# Autodesk Inventor assembly: drive_parts_assembly_z
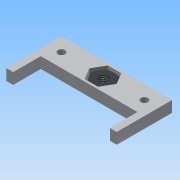
[picture p0: Inventor's stored thumbnail of the model, 180x180]
Saved by Autodesk Inventor 2015 (Build 190159000, 159)
## iProperties
Created: 2014-09-02
Part Number: drive_parts_assembly_z
Document SubType Name: Assembly
Designer: shohei
Author: shohei
## Documents named in this file (3)
- C:\Users\shohei\Documents\Inventor\PlasmaCNCrev3\Workspaces\Workspace\drive_parts_assembly_z.iam
- C:\Users\shohei\Documents\Inventor\PlasmaCNCrev3\Workspaces\Workspace\main\M8_driving_nut.ipt
- C:\Users\shohei\Documents\Inventor\PlasmaCNCrev3\Workspaces\Workspace\main\drive_support.ipt
## Components (2 placed, 2 different names)
1. M8_driving_nut:1 — Flush:1, Angle:1
2. drive_support:1 — Flush:1, Angle:1
## Relationships (2: Flush 1, Angle 1)
- Flush:1: M8_driving_nut:1 ↔ drive_support:1
- Angle:1 (0 deg): M8_driving_nut:1 ↔ drive_support:1
